# Autodesk Inventor assembly: Peep
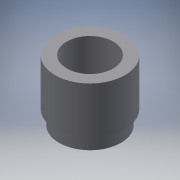
[picture p0: Inventor's stored thumbnail of the model, 180x180]
Saved by Autodesk Inventor 2018 (Build 220112000, 112)
## iProperties
Created: 2020-03-27
Part Number: Peep
Document SubType Name: Assembly
Designer: emile
Author: emile
## Documents named in this file (3)
- C:\Users\emile\OneDrive\Documents\Inventor\Respirator\Peep\Peep.iam
- C:\Users\emile\OneDrive\Documents\Inventor\Respirator\Peep\Diaphragm.iam
- C:\Users\emile\OneDrive\Documents\Inventor\Respirator\Peep\Tube.ipt
## Components (2 placed, 2 different names)
1. Diaphragm:1 [sub-assembly] — Mate:1, Tangent:1
2. Tube:1 — Mate:1, Mate:3, Mate:4, Flush:1, Tangent:1
## Relationships (5: Mate 3, Flush 1, Tangent 1)
- Mate:1: Diaphragm:1 ↔ Tube:1
- Mate:3: Tube:1
- Mate:4: Tube:1
- Flush:1: Tube:1
- Tangent:1: Diaphragm:1 ↔ Tube:1
